# Autodesk Inventor assembly: ADSK-MH-10014
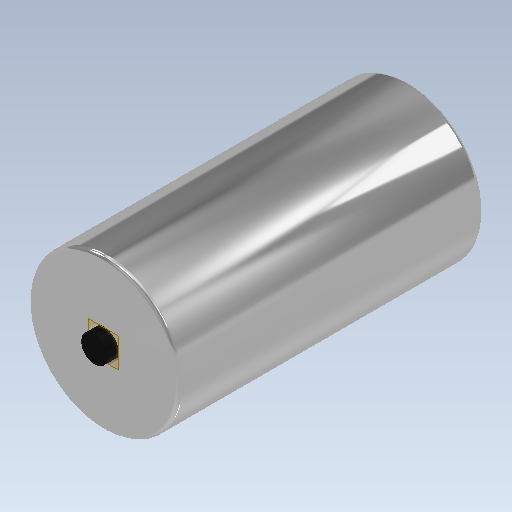
[picture p0: Inventor's stored thumbnail of the model, 512x512]
Saved by Autodesk Inventor 2021.1 (Build 251245010, 245A)
## iProperties
Created: 2008-03-10
Part Number: ADSK-MH-10014
Document SubType Name: Assembly
Designer: R.O'mahony
Description: Small Roller Assembly
Engineer: Demir Ali
Checked By: Demir Ali
Company: Autodesk Ltd
Author: R.O'mahony
Keywords: Roller Conveyor
Revision Number: A
## Documents named in this file (3)
- C:\Users\peter\source\repos\InventorDA-FLC\Dataset\Discharge Conveyor\ADSK-MH-10014.iam
- C:\Users\peter\source\repos\InventorDA-FLC\Dataset\Discharge Conveyor\ADSK-MH-10015.ipt
- C:\Users\peter\source\repos\InventorDA-FLC\Dataset\Discharge Conveyor\ADSK-MH-10016.ipt
## Components (2 placed, 2 different names)
1. Roller_bar — Flush:1
2. Roller — Flush:1
## Relationships (1: Flush 1)
- Flush:1: Roller_bar ↔ Roller
